# Autodesk Inventor assembly: 6P Sprocket
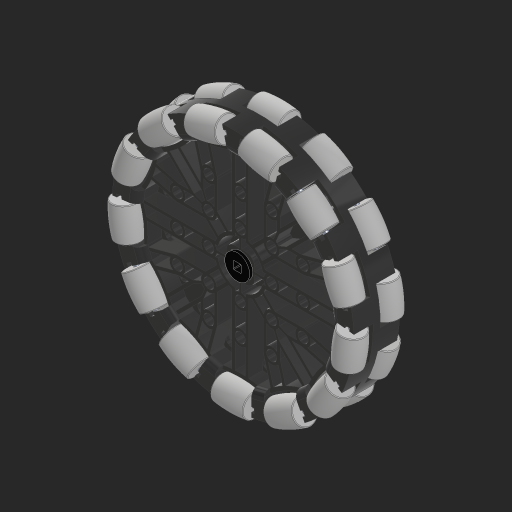
[picture p0: Inventor's stored thumbnail of the model, 512x512]
Saved by Autodesk Inventor 2023 (Build 270158000, 158)
## iProperties
Created: 2022-08-02
Part Number: 6P Sprocket
Document SubType Name: Assembly
Designer: ylu12
Author: ylu12
## Documents named in this file (4)
- C:\Users\ylu12\Documents\GitHub\VEX-CAD-Inventor\Motion\Wheels\Omni Wheel\4 Omni AS, Square.iam
- C:\Users\ylu12\Documents\GitHub\VEX-CAD-Inventor\Motion\Wheels\Reference Files\4 Omni Antistatic.ipt
- C:\Users\ylu12\Documents\GitHub\VEX-CAD-Inventor\Motion\Insert Square.ipt
- C:\Users\ylu12\Documents\GitHub\VEX-CAD-Inventor\Motion\Wheels\Omni Wheel.iam
## Components (3 placed, 3 different names)
1. 4 Omni Antistatic
2. Square 1 — Mate:17, Flush:10, Flush:11
3. Square 2 — Flush:9, Flush:10, Flush:11, Mate:18, Angle:1
## Relationships (9: Flush 4, Mate 4, Angle 1)
- [Flush]: 4 Omni Antistatic
- [Mate]: 4 Omni Antistatic
- [Mate]: 4 Omni Antistatic
- Flush:9 (6.35 mm): Square 2
- Mate:17 (6.35 mm): Square 1
- Flush:10: Square 1 ↔ Square 2
- Flush:11: Square 1 ↔ Square 2
- Mate:18: Square 2
- Angle:1 (0 deg): Square 2
## Named parameters: HalfWheelWidth = 6.35 mm
